# Autodesk Inventor assembly: V1Indexers
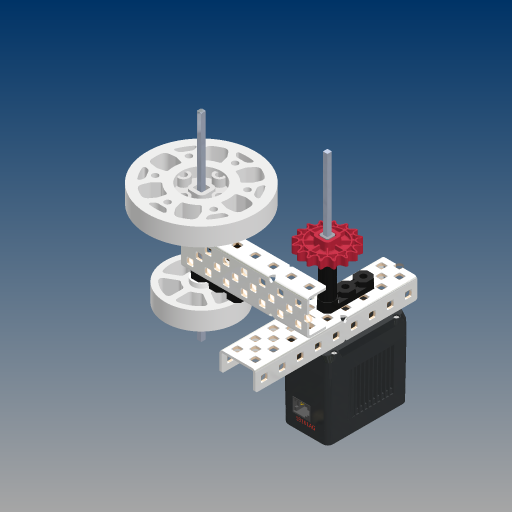
[picture p0: Inventor's stored thumbnail of the model, 512x512]
Saved by Autodesk Inventor 2023 (Build 270158000, 158)
## iProperties
Created: 2023-07-14
Part Number: V1Indexers
Document SubType Name: Assembly
Designer: eddie
Author: eddie
## Documents named in this file (22)
- C:\Users\eddie\Documents\81208X-Over-Under-CAD\V1\V1Indexers.iam
- C:\Users\eddie\Documents\81208X-Over-Under-CAD\VEX-CAD-Inventor-1.4.0\Structure\C Channel\Aluminum 1x2x1\Alu C 1x2x1x9.ipt
- C:\Users\eddie\Documents\81208X-Over-Under-CAD\VEX-CAD-Inventor-1.4.0\Motion\Shaft LS\Bearing Flat.ipt
- C:\Users\eddie\Documents\81208X-Over-Under-CAD\VEX-CAD-Inventor-1.4.0\Structure\C Channel\Aluminum 1x2x1\Alu C 1x2x1x7.ipt
- C:\Users\eddie\Documents\81208X-Over-Under-CAD\VEX-CAD-Inventor-1.4.0\Electronics\V5 Motor.ipt
- C:\Users\eddie\Documents\81208X-Over-Under-CAD\VEX-CAD-Inventor-1.4.0\Motion\Shaft LS\Shaft LS.ipt
- C:\Users\eddie\Documents\81208X-Over-Under-CAD\VEX-CAD-Inventor-1.4.0\Motion\Spacers\Spacer Nylon .375 OD\NSpacer .375 OD x .500.ipt
- C:\Users\eddie\Documents\81208X-Over-Under-CAD\VEX-CAD-Inventor-1.4.0\Motion\Spacers\Spacer Nylon .375 OD.ipt
- C:\Users\eddie\Documents\81208X-Over-Under-CAD\VEX-CAD-Inventor-1.4.0\Motion\Sprockets\6P Sprocket\6P 16T Sprocket, Square.iam
- C:\Users\eddie\Documents\81208X-Over-Under-CAD\VEX-CAD-Inventor-1.4.0\Motion\Sprockets\6P Sprocket.iam
- C:\Users\eddie\Documents\81208X-Over-Under-CAD\VEX-CAD-Inventor-1.4.0\Motion\Shaft LS\Shaft LS\Shaft LS 3.5.ipt
- C:\Users\eddie\Documents\81208X-Over-Under-CAD\VEX-CAD-Inventor-1.4.0\Motion\Shaft LS\Shaft LS\Shaft LS 5.5.ipt
- C:\Users\eddie\Documents\81208X-Over-Under-CAD\VEX-CAD-Inventor-1.4.0\Motion\Sprockets\6P Sprocket\6P 8T Sprocket, Square.iam
- C:\Users\eddie\Documents\81208X-Over-Under-CAD\VEX-CAD-Inventor-1.4.0\Motion\Spacers\Spacer Nylon .500 OD\NSpacer White .500 OD x .125.ipt
- C:\Users\eddie\Documents\81208X-Over-Under-CAD\VEX-CAD-Inventor-1.4.0\Motion\Spacers\Spacer Nylon .500 OD.ipt
- C:\Users\eddie\Documents\81208X-Over-Under-CAD\VEX-CAD-Inventor-1.4.0\Motion\Wheels\Flex Wheels\2.000 Flex Wheel\2.000 30A .500.ipt
- C:\Users\eddie\Documents\81208X-Over-Under-CAD\VEX-CAD-Inventor-1.4.0\Motion\Wheels\Flex Wheels\2.000 Flex Wheel.ipt
- C:\Users\eddie\Documents\81208X-Over-Under-CAD\VEX-CAD-Inventor-1.4.0\Motion\Gears\HS Gear\HS 12T Gear, Square.iam
- C:\Users\eddie\Documents\81208X-Over-Under-CAD\VEX-CAD-Inventor-1.4.0\Motion\Gears\HS Gear.iam
- C:\Users\eddie\Documents\81208X-Over-Under-CAD\VEX-CAD-Inventor-1.4.0\Motion\Wheels\Flex Wheels\3.000 Flex Wheel\3.000 30A .500.ipt
- C:\Users\eddie\Documents\81208X-Over-Under-CAD\VEX-CAD-Inventor-1.4.0\Motion\Wheels\Flex Wheels\3.000 Flex Wheel.ipt
- C:\Users\eddie\Documents\81208X-Over-Under-CAD\Custom-parts\36T HS Gear Insert_MIR.ipt
## Components (17 placed, 14 different names)
1. Alu C 1x2x1x9:1 — Insert:1, Insert:2
2. Bearing Flat:1 — Insert:1, Insert:5, Insert:13, Insert:14
3. Alu C 1x2x1x7:1 — Insert:2, Insert:11, Insert:12, Insert:17, Insert:20
4. V5 Motor:1 — Insert:5
5. Shaft LS 5.5:2
6. Bearing Flat:2 — Insert:11, Insert:12, Insert:19
7. Shaft LS 3.5:3 — Insert:13
8. NSpacer .375 OD x .500:3 — Insert:14, Insert:15
9. NSpacer .375 OD x .500:4 — Insert:15, Insert:16
10. 6P 16T Sprocket, Square:2 [sub-assembly] — Insert:16
11. 6P 8T Sprocket, Square:3 [sub-assembly] — Insert:17, Insert:39
12. NSpacer White .500 OD x .125:1 — Insert:19, Insert:21, Insert:22
13. Bearing Flat:3 — Insert:20
14. 2.000 30A .500:1 — Insert:22
15. HS 12T Gear, Square:1 [sub-assembly] — Insert:21
16. 3.000 30A .500:2 — Insert:39
17. 36T HS Gear Insert_MIR:1
## Relationships (15: Insert 15)
- Insert:1: Alu C 1x2x1x9:1 ↔ Bearing Flat:1
- Insert:2: Alu C 1x2x1x9:1 ↔ Alu C 1x2x1x7:1
- Insert:5: Bearing Flat:1 ↔ V5 Motor:1
- Insert:11: Alu C 1x2x1x7:1 ↔ Bearing Flat:2
- Insert:12: Alu C 1x2x1x7:1 ↔ Bearing Flat:2
- Insert:13: Bearing Flat:1 ↔ Shaft LS 3.5:3
- Insert:14: Bearing Flat:1 ↔ NSpacer .375 OD x .500:3
- Insert:15: NSpacer .375 OD x .500:3 ↔ NSpacer .375 OD x .500:4
- Insert:16: NSpacer .375 OD x .500:4 ↔ 6P 16T Sprocket, Square:2
- Insert:17: Alu C 1x2x1x7:1 ↔ 6P 8T Sprocket, Square:3
- Insert:19: Bearing Flat:2 ↔ NSpacer White .500 OD x .125:1
- Insert:20: Alu C 1x2x1x7:1 ↔ Bearing Flat:3
- Insert:21: NSpacer White .500 OD x .125:1 ↔ HS 12T Gear, Square:1
- Insert:22: NSpacer White .500 OD x .125:1 ↔ 2.000 30A .500:1
- Insert:39: 6P 8T Sprocket, Square:3 ↔ 3.000 30A .500:2
